# Autodesk Inventor assembly: subassembly_jar_jarcone
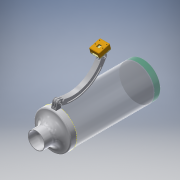
[picture p0: Inventor's stored thumbnail of the model, 180x180]
Saved by Autodesk Inventor 2019 (Build 230136000, 136)
## iProperties
Created: 2019-01-23
Part Number: subassembly_jar_jarcone
Document SubType Name: Assembly
Designer: jmc
Author: jmc
## Documents named in this file (3)
- C:\Users\l0086\Desktop\Models\CatFeeder\version4 (auger)\subassembly_jar_jarcone_gopro.iam
- C:\Users\l0086\Desktop\Models\CatFeeder\Jar\Jar.ipt
- C:\Users\l0086\Desktop\Models\CatFeeder\JarCone\version3\cone_gopro_assembly.iam
## Components (2 placed, 2 different names)
1. Jar:1 — Rigid:1
2. cone_gopro_assembly:1 [sub-assembly] — Rigid:1
## Relationships (1: WeldJoint 1)
- Rigid:1 [WeldJoint]: Jar:1 ↔ cone_gopro_assembly:1
